# Autodesk Inventor assembly: damascusCoverAssembly
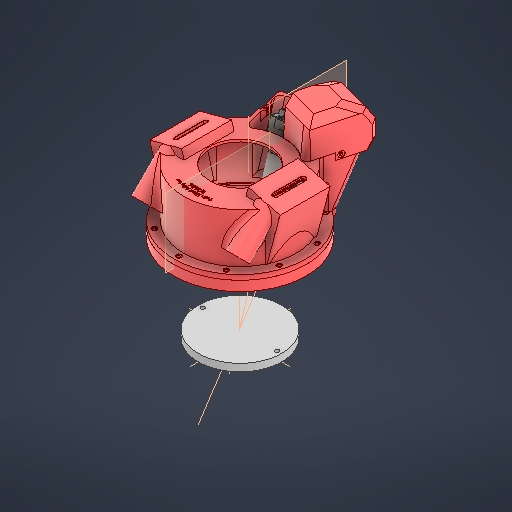
[picture p0: Inventor's stored thumbnail of the model, 512x512]
Saved by Autodesk Inventor 2026.2 (Build 302298000, 298)
## iProperties
Created: 2026-05-01
Part Number: damascusCoverAssembly
Document SubType Name: Assembly
Designer: mayhe
Author: mayhe
## Documents named in this file (12)
- C:\Users\mayhe\OneDrive\Documents\GitHub\In-situ-monitoring-of-powder-bed-fusion-additive-manufacturing\system_development\Damascus\V0.4\hardware development\damascusCoverAssembly.iam
- C:\Users\mayhe\OneDrive\Documents\GitHub\In-situ-monitoring-of-powder-bed-fusion-additive-manufacturing\system_development\Damascus\V0.4\hardware development\Parts\12mm Cover.ipt
- C:\Users\mayhe\OneDrive\Documents\GitHub\In-situ-monitoring-of-powder-bed-fusion-additive-manufacturing\system_development\Damascus\V0.4\hardware development\Parts\Build Plate with 35mm FOV Sketch.ipt
- C:\Users\mayhe\OneDrive\Documents\GitHub\In-situ-monitoring-of-powder-bed-fusion-additive-manufacturing\system_development\Damascus\V0.4\hardware development\Parts\sealRing.ipt
- C:\Users\mayhe\OneDrive\Documents\GitHub\In-situ-monitoring-of-powder-bed-fusion-additive-manufacturing\system_development\Damascus\V0.4\hardware development\Parts\Xi-410-Camera-with-29°-x-18°-Lens\Xi 410 Camera with 29° x.iam
- C:\Users\mayhe\OneDrive\Documents\GitHub\In-situ-monitoring-of-powder-bed-fusion-additive-manufacturing\system_development\Damascus\V0.4\hardware development\Parts\Optical Camera\Camera with 35mm.iam
- C:\Users\mayhe\OneDrive\Documents\GitHub\In-situ-monitoring-of-powder-bed-fusion-additive-manufacturing\system_development\Damascus\V0.4\hardware development\Parts\Antireflective Glass.ipt
- C:\Users\mayhe\OneDrive\Documents\GitHub\In-situ-monitoring-of-powder-bed-fusion-additive-manufacturing\system_development\Damascus\V0.4\hardware development\Parts\adapter-optical.ipt
- C:\Users\mayhe\OneDrive\Documents\GitHub\In-situ-monitoring-of-powder-bed-fusion-additive-manufacturing\system_development\Damascus\V0.4\hardware development\Parts\twinHead - adapter - new socket.ipt
- C:\Users\mayhe\OneDrive\Documents\GitHub\In-situ-monitoring-of-powder-bed-fusion-additive-manufacturing\system_development\Damascus\V0.4\hardware development\Parts\twinheadLid.ipt
- C:\Users\mayhe\OneDrive\Documents\GitHub\In-situ-monitoring-of-powder-bed-fusion-additive-manufacturing\system_development\Damascus\V0.4\hardware development\Parts\Event Camera\Triton2_asm.iam
- C:\Users\mayhe\OneDrive\Documents\GitHub\In-situ-monitoring-of-powder-bed-fusion-additive-manufacturing\system_development\Damascus\V0.4\hardware development\Parts\adapter-event.ipt
## Components (11 placed, 11 different names)
1. 12mm Cover:1 — Rotational:1, Rotational:2
2. Build Plate with 35mm FOV Sketch:1 — Rotational:1
3. sealRing:1 — Rotational:2, Rotational:5
4. Xi 410 Camera with 29° x:1 [sub-assembly] — Rotational:15
5. Antireflective Glass:1 — Rotational:5
6. twinHead - adapter - new socket:1 — Rotational:15, Rotational:16, Mate:1, Mate:2, Rotational:18
7. twinheadLid:1 — Mate:1, Mate:2
8. Camera with 35mm:1 [sub-assembly] — Rotational:17
9. adapter-optical:1 — Rotational:16, Rotational:17
10. Triton2_asm:1 [sub-assembly] — Rotational:19
11. adapter-event:1 — Rotational:18, Rotational:19
## Relationships (10: RevoluteJoint 8, Mate 2)
- Rotational:1 [RevoluteJoint] (-150 mm): 12mm Cover:1 ↔ Build Plate with 35mm FOV Sketch:1
- Rotational:2 [RevoluteJoint]: 12mm Cover:1 ↔ sealRing:1
- Rotational:5 [RevoluteJoint]: sealRing:1 ↔ Antireflective Glass:1
- Rotational:15 [RevoluteJoint]: Xi 410 Camera with 29° x:1 ↔ twinHead - adapter - new socket:1
- Rotational:16 [RevoluteJoint]: twinHead - adapter - new socket:1 ↔ adapter-optical:1
- Rotational:17 [RevoluteJoint]: Camera with 35mm:1 ↔ adapter-optical:1
- Mate:1 (0.2 mm): twinHead - adapter - new socket:1 ↔ twinheadLid:1
- Mate:2: twinHead - adapter - new socket:1 ↔ twinheadLid:1
- Rotational:18 [RevoluteJoint]: twinHead - adapter - new socket:1 ↔ adapter-event:1
- Rotational:19 [RevoluteJoint]: Triton2_asm:1 ↔ adapter-event:1
